# Autodesk Inventor assembly: PocketNC_Workpiece_Base
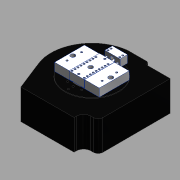
[picture p0: Inventor's stored thumbnail of the model, 180x180]
Saved by Autodesk Inventor 2017 (Build 210142000, 142)
## iProperties
Created: 2018-06-05
Part Number: PocketNC_Workpiece_Base
Document SubType Name: Assembly
Designer: Jarrett
Author: Jarrett
## Documents named in this file (6)
- C:\Users\Jarrett\Desktop\Research Summer 2018\PocketNC_Workpiece_Base.iam
- C:\Users\Jarrett\Desktop\Research Summer 2018\PocketNC_Vise_Backing_Plate.ipt
- C:\Users\Jarrett\Desktop\Research Summer 2018\PocketNC_Vise_part2.ipt
- C:\Users\Jarrett\Desktop\Research Summer 2018\PocketNC_Vise_part1.ipt
- C:\Users\Jarrett\Desktop\Research Summer 2018\PocketNC_Workpiece_Y_axis_rotation.ipt
- C:\Users\Jarrett\Desktop\Research Summer 2018\PocketNC_Workpiece_Z_axis_rotation.ipt
## Components (5 placed, 5 different names)
1. PocketNC_Vise_Backing_Plate:1 — Mate:2, Mate:3, Flush:1, Mate:4, Angle:1, Mate:6, Mate:7
2. PocketNC_Vise_part2:1 — Mate:2, Mate:4, Angle:1, Angle:3, Mate:5
3. PocketNC_Vise_part1:1 — Angle:3, Mate:5
4. PocketNC_Workpiece_Y_axis_rotation:1 — Mate:6, Mate:7, Mate:8, Mate:9
5. PocketNC_Workpiece_Z_axis_rotation:1 — Mate:8, Mate:9
## Relationships (11: Mate 8, Angle 2, Flush 1)
- Mate:2: PocketNC_Vise_Backing_Plate:1 ↔ PocketNC_Vise_part2:1
- Mate:3: PocketNC_Vise_Backing_Plate:1
- Flush:1: PocketNC_Vise_Backing_Plate:1
- Mate:4: PocketNC_Vise_Backing_Plate:1 ↔ PocketNC_Vise_part2:1
- Angle:1 (180 deg): PocketNC_Vise_Backing_Plate:1 ↔ PocketNC_Vise_part2:1
- Angle:3 (0 deg): PocketNC_Vise_part2:1 ↔ PocketNC_Vise_part1:1
- Mate:5: PocketNC_Vise_part2:1 ↔ PocketNC_Vise_part1:1
- Mate:6: PocketNC_Vise_Backing_Plate:1 ↔ PocketNC_Workpiece_Y_axis_rotation:1
- Mate:7: PocketNC_Vise_Backing_Plate:1 ↔ PocketNC_Workpiece_Y_axis_rotation:1
- Mate:8: PocketNC_Workpiece_Y_axis_rotation:1 ↔ PocketNC_Workpiece_Z_axis_rotation:1
- Mate:9: PocketNC_Workpiece_Y_axis_rotation:1 ↔ PocketNC_Workpiece_Z_axis_rotation:1
